# Autodesk Inventor assembly: ASY DUMMY TANK
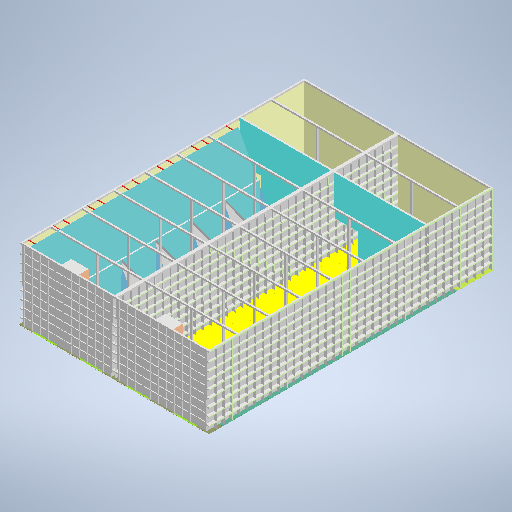
[picture p0: Inventor's stored thumbnail of the model, 512x512]
Saved by Autodesk Inventor 2026 (Build 300175000, 175)
## iProperties
Created: 2026-07-16
Part Number: ASY DUMMY TANK
Document SubType Name: Assembly
Designer: admin
Author: admin
## Documents named in this file (4)
- C:\Users\user\Documents\Inventor\GBK-Gubkinskiy\dummy\ASY DUMMY TANK.iam
- C:\Users\user\Documents\Inventor\GBK-Gubkinskiy\GBK overall model.ipt
- C:\Users\user\Documents\Inventor\GBK-Gubkinskiy\dummy\Pocket.ipt
- C:\Users\user\Documents\Inventor\GBK-Gubkinskiy\090 ASY bottom.iam
## Components (8 placed, 3 different names)
1. GBK overall model:1 — Совмещение:1, Совмещение:2, Заподлицо:1, Совмещение:3, Заподлицо:2, Заподлицо:3
2. 090 ASY bottom:1 [sub-assembly] — Совмещение:3, Заподлицо:2, Заподлицо:3
3. Pocket:1 — Совмещение:1, Совмещение:2, Заподлицо:1
4. Pocket:2
5. Pocket:3
6. Pocket:4
7. Pocket:5
8. Pocket:6
## Component patterns: (6 elements, first: Pocket:1)
## Relationships (6: Mate 3, Flush 3)
- Совмещение:1 [Mate]: GBK overall model:1 ↔ Pocket:1
- Совмещение:2 [Mate]: GBK overall model:1 ↔ Pocket:1
- Заподлицо:1 [Flush]: GBK overall model:1 ↔ Pocket:1
- Совмещение:3 [Mate]: GBK overall model:1 ↔ 090 ASY bottom:1
- Заподлицо:2 [Flush] (-50 mm): GBK overall model:1 ↔ 090 ASY bottom:1
- Заподлицо:3 [Flush] (-50 mm): GBK overall model:1 ↔ 090 ASY bottom:1
